# Autodesk Inventor assembly: VİDA_MİLİ2
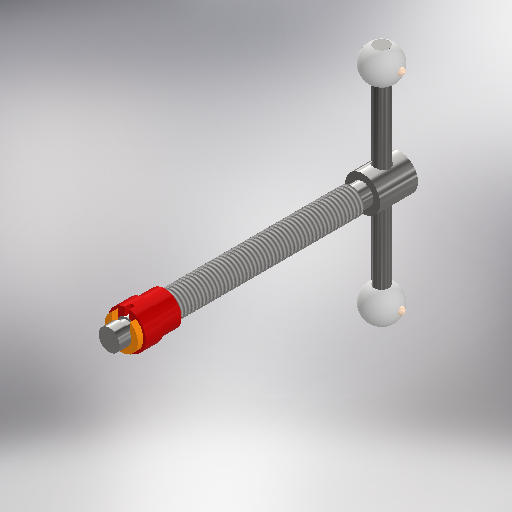
[picture p0: Inventor's stored thumbnail of the model, 512x512]
Saved by Autodesk Inventor 2025.4 (Build 294407000, 407)
## iProperties
Created: 2026-06-22
Part Number: VİDA_MİLİ2
Document SubType Name: Assembly
Designer: win10
Author: win10
## Documents named in this file (7)
- C:\Users\yigithan\Desktop\mengene\VİDA_MİLİ2.iam
- C:\Users\yigithan\Desktop\mengene\parca4.ipt
- C:\Users\yigithan\Desktop\mengene\parca7.ipt
- C:\Users\yigithan\Desktop\mengene\parca8.ipt
- C:\Users\yigithan\Desktop\mengene\parça3.ipt
- C:\Users\yigithan\Desktop\mengene\parça5.ipt
- C:\Users\yigithan\Desktop\mengene\parça6.ipt
## Components (8 placed, 6 different names)
1. parca4:1 — Mate:1, Mate:2, Mate:3, Mate:4, Mate:5
2. parca7:1 — Mate:2, Mate:3, Mate:6, Mate:7, Mate:10
3. parca8:1 — Mate:6, Mate:7
4. parça3:1 — Mate:1, Insert:1, Insert:2
5. parça5:1 — Insert:1
6. parça6:1 — Insert:2
7. parca7:2 — Mate:4, Mate:5, Mate:8, Mate:9
8. parca8:2 — Mate:8, Mate:9
## Relationships (12: Mate 10, Insert 2)
- Mate:1: parca4:1 ↔ parça3:1
- Mate:2: parca4:1 ↔ parca7:1
- Mate:3: parca4:1 ↔ parca7:1
- Mate:4: parca4:1 ↔ parca7:2
- Mate:5: parca4:1 ↔ parca7:2
- Mate:6: parca7:1 ↔ parca8:1
- Mate:7: parca7:1 ↔ parca8:1
- Mate:8: parca7:2 ↔ parca8:2
- Mate:9: parca7:2 ↔ parca8:2
- Mate:10 (-65.09 mm): parca7:1
- Insert:1: parça3:1 ↔ parça5:1
- Insert:2: parça3:1 ↔ parça6:1
